# Autodesk Inventor assembly: lowerArm
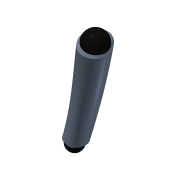
[picture p0: Inventor's stored thumbnail of the model, 180x180]
Saved by Autodesk Inventor 2018 (Build 220112000, 112)
## iProperties
Created: 2020-03-01
Part Number: lowerArm
Document SubType Name: Assembly
Designer: Matt
Author: Matt
## Documents named in this file (2)
- C:\Users\Matt\robot\multibodySim\human\Corpo Humano - ADEBOTT Projetos\lowerArm.iam
- C:\Users\Matt\robot\multibodySim\human\Corpo Humano - ADEBOTT Projetos\01.02.02.02 - Antebraço direito.ipt
## Components (1 placed, 1 different names)
1. 01.02.02.02 - Antebraço direito:1 — Flush:1, Flush:2, Flush:3
## Relationships (3: Flush 3)
- Flush:1 (-1125 mm): 01.02.02.02 - Antebraço direito:1
- Flush:2 (219 mm): 01.02.02.02 - Antebraço direito:1
- Flush:3 (65 mm): 01.02.02.02 - Antebraço direito:1
